# Autodesk Inventor assembly: DPLX_A004_VIPE_Lab
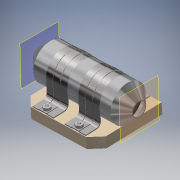
[picture p0: Inventor's stored thumbnail of the model, 180x180]
Saved by Autodesk Inventor 2018 (Build 220112000, 112)
## iProperties
Created: 2018-07-19
Part Number: DPLX_A004_VIPE_Lab
Document SubType Name: Assembly
Designer: DPLXuser
Author: DPLXuser
## Documents named in this file (12)
- C:\Users\DPLXuser\Documents\Michael Schwab\SPARK CAD Files\DPLX_A004_VIPE_Lab.iam
- C:\Users\DPLXuser\Documents\Michael Schwab\SPARK CAD Files\DPLX_P030_VIPE Insulation Bottom.ipt
- C:\Users\DPLXuser\Documents\Michael Schwab\SPARK CAD Files\DPLX_P031_VIPE Insulation Top.ipt
- C:\Users\DPLXuser\Documents\Michael Schwab\SPARK CAD Files\DPLX_P032_VIPE Insulation Middle.ipt
- C:\Users\DPLXuser\Documents\Michael Schwab\SPARK CAD Files\92010A787_PASSIVATED 18-8 SS PHILLIPS FLAT HEAD SCREW.ipt
- C:\Users\DPLXuser\Documents\Michael Schwab\SPARK CAD Files\92010A122_METRIC 18-8 SS FLAT HEAD PHIL MACHINE SCREW.ipt
- C:\Users\DPLXuser\Documents\Michael Schwab\SPARK CAD Files\9429T360_STEEL CLAMP.ipt
- C:\Users\DPLXuser\Documents\Michael Schwab\SPARK CAD Files\DPLX_P026_VIPE _Transformer.ipt
- C:\Users\DPLXuser\Documents\Michael Schwab\SPARK CAD Files\DPLX_P034_RPS VIPE Viton Insualtion.ipt
- C:\Users\DPLXuser\Documents\Michael Schwab\SPARK CAD Files\DPLX_P008_Wire_Mesh_Sleeve_Trans.ipt
- C:\Users\DPLXuser\Documents\Michael Schwab\SPARK CAD Files\DPLX_P009_Wire_Mesh_reducer_Trans.ipt
- C:\Users\DPLXuser\Documents\Michael Schwab\SPARK CAD Files\91828A211_TYPE 18-8 STAINLESS STEEL HEX NUT.ipt
## Components (22 placed, 11 different names)
1. DPLX_P030_VIPE Insulation Bottom:1 — Insert:9, Insert:10
2. DPLX_P031_VIPE Insulation Top:1 — Insert:11, Insert:12, Insert:13, Insert:14, Insert:15, Insert:16, Mate:1
3. DPLX_P032_VIPE Insulation Middle:1 — Insert:1, Insert:2, Insert:3, Insert:4, Insert:5, Insert:6, Insert:7, Insert:8, Insert:9, Insert:10, Insert:11, Insert:12
4. 92010A787_PASSIVATED 18-8 SS PHILLIPS FLAT HEAD SCREW:1 — Insert:1
5. 92010A787_PASSIVATED 18-8 SS PHILLIPS FLAT HEAD SCREW:2 — Insert:3
6. 92010A787_PASSIVATED 18-8 SS PHILLIPS FLAT HEAD SCREW:3 — Insert:4
7. 92010A787_PASSIVATED 18-8 SS PHILLIPS FLAT HEAD SCREW:4 — Insert:2
8. 92010A122_METRIC 18-8 SS FLAT HEAD PHIL MACHINE SCREW:1 — Insert:8
9. 92010A122_METRIC 18-8 SS FLAT HEAD PHIL MACHINE SCREW:2 — Insert:7
10. 92010A122_METRIC 18-8 SS FLAT HEAD PHIL MACHINE SCREW:3 — Insert:6
11. 92010A122_METRIC 18-8 SS FLAT HEAD PHIL MACHINE SCREW:4 — Insert:5
12. 9429T360_STEEL CLAMP:1 — Insert:15, Insert:16, Insert:22, Insert:25
13. 9429T360_STEEL CLAMP:2 — Insert:13, Insert:14, Insert:18, Insert:23, Insert:24
14. DPLX_P034_RPS VIPE Viton Insualtion:1 — Insert:17, Insert:18, Insert:19
15. DPLX_P026_VIPE _Transformer:1 — Insert:17, Mate:1
16. DPLX_P008_Wire_Mesh_Sleeve_Trans:1 — Insert:19, Insert:20, Insert:21
17. DPLX_P009_Wire_Mesh_reducer_Trans:1 — Insert:21
18. DPLX_P009_Wire_Mesh_reducer_Trans:2 — Insert:20
19. 91828A211_TYPE 18-8 STAINLESS STEEL HEX NUT:1 — Insert:24
20. 91828A211_TYPE 18-8 STAINLESS STEEL HEX NUT:2 — Insert:25
21. 91828A211_TYPE 18-8 STAINLESS STEEL HEX NUT:3 — Insert:23
22. 91828A211_TYPE 18-8 STAINLESS STEEL HEX NUT:4 — Insert:22
## Relationships (26: Insert 25, Mate 1)
- Insert:1: DPLX_P032_VIPE Insulation Middle:1 ↔ 92010A787_PASSIVATED 18-8 SS PHILLIPS FLAT HEAD SCREW:1
- Insert:2: DPLX_P032_VIPE Insulation Middle:1 ↔ 92010A787_PASSIVATED 18-8 SS PHILLIPS FLAT HEAD SCREW:4
- Insert:3: DPLX_P032_VIPE Insulation Middle:1 ↔ 92010A787_PASSIVATED 18-8 SS PHILLIPS FLAT HEAD SCREW:2
- Insert:4: DPLX_P032_VIPE Insulation Middle:1 ↔ 92010A787_PASSIVATED 18-8 SS PHILLIPS FLAT HEAD SCREW:3
- Insert:5: DPLX_P032_VIPE Insulation Middle:1 ↔ 92010A122_METRIC 18-8 SS FLAT HEAD PHIL MACHINE SCREW:4
- Insert:6: DPLX_P032_VIPE Insulation Middle:1 ↔ 92010A122_METRIC 18-8 SS FLAT HEAD PHIL MACHINE SCREW:3
- Insert:7: DPLX_P032_VIPE Insulation Middle:1 ↔ 92010A122_METRIC 18-8 SS FLAT HEAD PHIL MACHINE SCREW:2
- Insert:8: DPLX_P032_VIPE Insulation Middle:1 ↔ 92010A122_METRIC 18-8 SS FLAT HEAD PHIL MACHINE SCREW:1
- Insert:9: DPLX_P030_VIPE Insulation Bottom:1 ↔ DPLX_P032_VIPE Insulation Middle:1
- Insert:10: DPLX_P030_VIPE Insulation Bottom:1 ↔ DPLX_P032_VIPE Insulation Middle:1
- Insert:11: DPLX_P031_VIPE Insulation Top:1 ↔ DPLX_P032_VIPE Insulation Middle:1
- Insert:12: DPLX_P031_VIPE Insulation Top:1 ↔ DPLX_P032_VIPE Insulation Middle:1
- Insert:13 (0.3302 mm): DPLX_P031_VIPE Insulation Top:1 ↔ 9429T360_STEEL CLAMP:2
- Insert:14 (0.3302 mm): DPLX_P031_VIPE Insulation Top:1 ↔ 9429T360_STEEL CLAMP:2
- Insert:15 (0.3302 mm): DPLX_P031_VIPE Insulation Top:1 ↔ 9429T360_STEEL CLAMP:1
- Insert:16 (0.3302 mm): DPLX_P031_VIPE Insulation Top:1 ↔ 9429T360_STEEL CLAMP:1
- Insert:17: DPLX_P034_RPS VIPE Viton Insualtion:1 ↔ DPLX_P026_VIPE _Transformer:1
- Insert:18 (-7.62 mm): 9429T360_STEEL CLAMP:2 ↔ DPLX_P034_RPS VIPE Viton Insualtion:1
- Mate:1: DPLX_P031_VIPE Insulation Top:1 ↔ DPLX_P026_VIPE _Transformer:1
- Insert:19 (-2.54 mm): DPLX_P034_RPS VIPE Viton Insualtion:1 ↔ DPLX_P008_Wire_Mesh_Sleeve_Trans:1
- Insert:20: DPLX_P008_Wire_Mesh_Sleeve_Trans:1 ↔ DPLX_P009_Wire_Mesh_reducer_Trans:2
- Insert:21: DPLX_P008_Wire_Mesh_Sleeve_Trans:1 ↔ DPLX_P009_Wire_Mesh_reducer_Trans:1
- Insert:22: 9429T360_STEEL CLAMP:1 ↔ 91828A211_TYPE 18-8 STAINLESS STEEL HEX NUT:4
- Insert:23: 9429T360_STEEL CLAMP:2 ↔ 91828A211_TYPE 18-8 STAINLESS STEEL HEX NUT:3
- Insert:24: 9429T360_STEEL CLAMP:2 ↔ 91828A211_TYPE 18-8 STAINLESS STEEL HEX NUT:1
- Insert:25: 9429T360_STEEL CLAMP:1 ↔ 91828A211_TYPE 18-8 STAINLESS STEEL HEX NUT:2
